# Autodesk Inventor assembly: Первая версия ноги
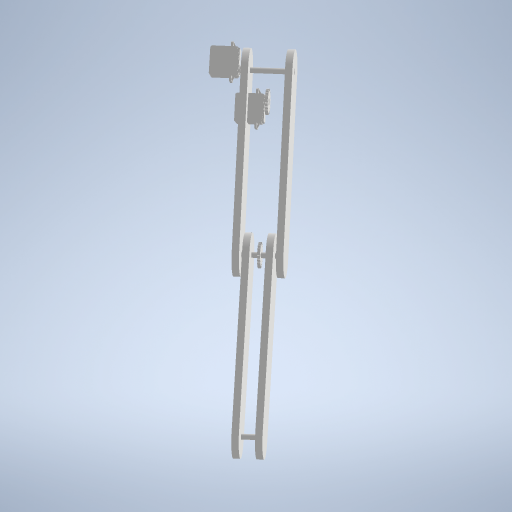
[picture p0: Inventor's stored thumbnail of the model, 512x512]
Saved by Autodesk Inventor 2023.2 (Build 272271000, 271)
## iProperties
Created: 2024-07-30
Part Number: Первая версия ноги
Document SubType Name: Assembly
Designer: End_Ways
Author: End_Ways
## Documents named in this file (7)
- C:\Users\End_Ways\Documents\МиниПес ЛРИМ\Первая версия ноги.iam
- C:\Users\End_Ways\Documents\МиниПес ЛРИМ\сервопривод DS3240.ipt
- C:\Users\End_Ways\Documents\МиниПес ЛРИМ\Вспомогательная деталь 2.ipt
- C:\Users\End_Ways\Documents\МиниПес ЛРИМ\Вспомогательная деталь 1.ipt
- C:\Users\End_Ways\Documents\МиниПес ЛРИМ\Вспомогательная деталь 3.ipt
- C:\Users\End_Ways\Documents\МиниПес ЛРИМ\Вспомогательная деталь 4.ipt
- C:\Users\End_Ways\Documents\МиниПес ЛРИМ\Рычаг.ipt
## Components (11 placed, 6 different names)
1. сервопривод DS3240:2 — С поворотом:2, Совмещение:1, Совмещение:2, Совмещение:3
2. Вспомогательная деталь 1:1 — С поворотом:2
3. Вспомогательная деталь 3:1 — Жесткий:1, С поворотом:5, С поворотом:6, Жесткий:4, Жесткий:5
4. Вспомогательная деталь 1:2 — Жесткий:1
5. Вспомогательная деталь 2:1 — С поворотом:4, Жесткий:2, Жесткий:3
6. сервопривод DS3240:3 — С поворотом:4
7. Вспомогательная деталь 4:1 — Жесткий:6
8. Рычаг:1 — Жесткий:2, С поворотом:6, Совмещение:1, Совмещение:2, Совмещение:3
9. Рычаг:2 — Жесткий:3, С поворотом:5
10. Рычаг:3 — Жесткий:4, Жесткий:6
11. Рычаг:4 — Жесткий:5
## Relationships (13: WeldJoint 6, RevoluteJoint 4, Mate 3)
- С поворотом:2 [RevoluteJoint]: сервопривод DS3240:2 ↔ Вспомогательная деталь 1:1
- Жесткий:1 [WeldJoint] (23 mm): Вспомогательная деталь 3:1 ↔ Вспомогательная деталь 1:2
- С поворотом:4 [RevoluteJoint]: Вспомогательная деталь 2:1 ↔ сервопривод DS3240:3
- Жесткий:2 [WeldJoint] (60 mm): Вспомогательная деталь 2:1 ↔ Рычаг:1
- Жесткий:3 [WeldJoint]: Вспомогательная деталь 2:1 ↔ Рычаг:2
- С поворотом:5 [RevoluteJoint]: Вспомогательная деталь 3:1 ↔ Рычаг:2
- С поворотом:6 [RevoluteJoint]: Вспомогательная деталь 3:1 ↔ Рычаг:1
- Жесткий:4 [WeldJoint] (-14 mm): Вспомогательная деталь 3:1 ↔ Рычаг:3
- Жесткий:5 [WeldJoint] (-14 mm): Вспомогательная деталь 3:1 ↔ Рычаг:4
- Жесткий:6 [WeldJoint]: Вспомогательная деталь 4:1 ↔ Рычаг:3
- Совмещение:1 [Mate] (-18 mm): сервопривод DS3240:2 ↔ Рычаг:1
- Совмещение:2 [Mate] (-38 mm): сервопривод DS3240:2 ↔ Рычаг:1
- Совмещение:3 [Mate] (-72 mm): сервопривод DS3240:2 ↔ Рычаг:1
